# Autodesk Inventor assembly: ZP3-T10BSJ10-B5
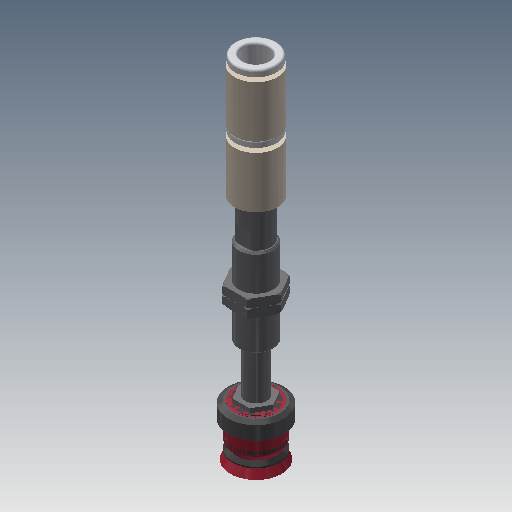
[picture p0: Inventor's stored thumbnail of the model, 512x512]
Saved by Autodesk Inventor 2019 (Build 230136000, 136)
## iProperties
Created: 2017-07-11
Part Number: ZP3-T10BSJ10-B5
Description: STEP AP214
Document SubType Name: Assembly
Designer: romanp
Title: ZP3-T10BSJ10-B5.step.step
Author: Windows User
Revision Number: ANY
## Documents named in this file (5)
- D:\DESKTOP\actual_github\3D\SMC_GRIP_SMALL\ZP3-T10BSJ10-B5.iam
- D:\DESKTOP\actual_github\3D\SMC_GRIP_SMALL\ZP3-T10BSJ10-B5.step_ZP3-B(4-10)_10.ipt
- D:\DESKTOP\actual_github\3D\SMC_GRIP_SMALL\ZP3-T10BSJ10-B5.step_T2AJ,AK,BJ,BK(3,6,10)-B5_T2AJ10-B5.ipt
- D:\DESKTOP\actual_github\3D\SMC_GRIP_SMALL\ZP10US.iam
- D:\DESKTOP\actual_github\3D\SMC_GRIP_SMALL\KQ2S06-M5A.iam
## Components (5 placed, 4 different names)
1. ZP3-T10BSJ10-B5.step_ZP3-B(4-10)_10_1
2. ZP3-T10BSJ10-B5.step_T2AJ,AK,BJ,BK(3,6,10)-B5_T2AJ10-B5_2 — Insert:1, Insert:2
3. ZP10US:1 [sub-assembly] — Insert:1
4. KQ2S06-M5A:1 [sub-assembly] — Insert:2, Insert:3
5. KQ2S06-M5A:2 [sub-assembly] — Insert:3
## Relationships (3: Insert 3)
- Insert:1: ZP3-T10BSJ10-B5.step_T2AJ,AK,BJ,BK(3,6,10)-B5_T2AJ10-B5_2 ↔ ZP10US:1
- Insert:2: ZP3-T10BSJ10-B5.step_T2AJ,AK,BJ,BK(3,6,10)-B5_T2AJ10-B5_2 ↔ KQ2S06-M5A:1
- Insert:3: KQ2S06-M5A:1 ↔ KQ2S06-M5A:2
